# Autodesk Inventor assembly: electrical board back
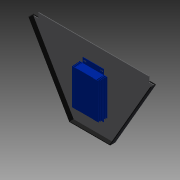
[picture p0: Inventor's stored thumbnail of the model, 180x180]
Saved by Autodesk Inventor 2012 (Build 160160000, 160)
## iProperties
Created: 2011-10-06
Part Number: electrical board back
Document SubType Name: Assembly
Designer: Antonella
Author: Antonella
## Documents named in this file (4)
- C:\Users\Antonella\Documents\GCC Robotics 2012 - Mechanical\Robot 2.0\Electrical\electrical board back.iam
- C:\Users\Antonella\Documents\GCC Robotics 2012 - Mechanical\Robot 2.0\Electrical\electrical board back.ipt
- C:\Users\Antonella\Documents\GCC Robotics 2012 - Mechanical\Robot 2.0\Electrical\Roboteq_HDC2450\Roboteq_HDC2450.ipt
- C:\Users\Antonella\Documents\GCC Robotics 2012 - Mechanical\Robot 2.0\Electrical\electronics board frame back.iam
## Components (3 placed, 3 different names)
1. electrical board back:1 — Mate:1, Flush:1, Flush:2, Mate:2, Flush:3, Mate:3
2. Roboteq_HDC2450:1 — Mate:1, Flush:1, Flush:2
3. electronics board frame back:1 [sub-assembly] — Mate:2, Flush:3, Mate:3
## Relationships (6: Mate 3, Flush 3)
- Mate:1: electrical board back:1 ↔ Roboteq_HDC2450:1
- Flush:1 (63.5 mm): electrical board back:1 ↔ Roboteq_HDC2450:1
- Flush:2: electrical board back:1 ↔ Roboteq_HDC2450:1
- Mate:2: electrical board back:1 ↔ electronics board frame back:1
- Flush:3: electrical board back:1 ↔ electronics board frame back:1
- Mate:3: electrical board back:1 ↔ electronics board frame back:1
